# Autodesk Inventor assembly: quadcopter
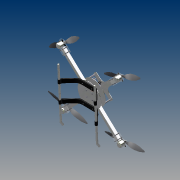
[picture p0: Inventor's stored thumbnail of the model, 180x180]
Saved by Autodesk Inventor 2011 SP1 (Build 150282100, 282)
## iProperties
Created: 2011-07-18
Part Number: quadcopter
Document SubType Name: Assembly
Designer: Nathan
Author: Nathan
## Documents named in this file (22)
- C:\Users\Nathan\Documents\Inventor\Quadcopter\quadcopter.iam
- C:\Users\Nathan\Documents\Inventor\Quadcopter\Arm.ipt
- C:\Users\Nathan\Documents\Inventor\Quadcopter\BaseTop.ipt
- C:\Users\Nathan\Documents\Inventor\Quadcopter\BaseBottom.ipt
- C:\Users\Nathan\Documents\Inventor\Quadcopter\MotorMount.iam
- C:\Users\Nathan\Documents\Inventor\Quadcopter\standoffiPart.ipt
- C:\Users\Nathan\Documents\Inventor\Quadcopter\standoffiPart-021.ipt
- C:\Users\Nathan\Documents\Inventor\Content Center Files\R2011\en-US\ANSI B18.6.3(26)\ANSI B18.6.3 - 8-32 UNC - 1.25(7).ipt
- C:\Users\Nathan\Documents\Inventor\Content Center Files\R2011\en-US\ANSI B18.6.3(26)\ANSI B18.6.3 - 8-32 UNC - 1.125(7).ipt
- C:\Users\Nathan\Documents\Inventor\Quadcopter\Imported Components\User Library-Arduino Mega\Assembly2.iam
- C:\Users\Nathan\Documents\Inventor\Quadcopter\LandingGear.iam
- C:\Users\Nathan\Documents\Inventor\Quadcopter\TopPlate.ipt
- C:\Users\Nathan\Documents\Inventor\Content Center Files\R2011\en-US\ANSI B18.6.3(26)\ANSI B18.6.3 - 8-32 UNC - 0.5(7).ipt
- C:\Users\Nathan\Documents\Inventor\Content Center Files\R2011\en-US\ANSI B18.6.3(26)\ANSI B18.6.3 - 4-40 UNC - 0.625(7).ipt
- C:\Users\Nathan\Documents\Inventor\Quadcopter\Motor.iam
- C:\Users\Nathan\Documents\Inventor\Quadcopter\propeller.iam
- C:\Users\Nathan\Documents\Inventor\Content Center Files\R2011\en-US\ANSI B18.6.3(26)\ANSI B18.6.3 - 6-32 UNC - 0.5625(7).ipt
- C:\Users\Nathan\Documents\Inventor\Quadcopter\PropProtector.ipt
- C:\Users\Nathan\Documents\Inventor\Content Center Files\R2011\en-US\ANSI B18.6.3(26)\ANSI B18.6.3 - 8-32 UNC - 1.375(7).ipt
- C:\Users\Nathan\Documents\Inventor\Content Center Files\R2011\en-US\ANSI B18.6.3(26)\ANSI B18.6.3 - 6-32 UNC - 0.5(7).ipt
- C:\Users\Nathan\Documents\Inventor\Quadcopter\Spacer_8-32.ipt
- C:\Users\Nathan\Documents\Inventor\Quadcopter\Spacer_4-40.ipt
## Components (58 placed, 20 different names)
1. Arm:1 — Mate:1, Mate:2, Mate:15, Flush:20, Mate:20, Flush:27, Mate:168, Mate:169
2. Arm:2 — Mate:5, Mate:6, Flush:21, Mate:21, Mate:38, Flush:25, Mate:160, Mate:161
3. Arm:3 — Mate:3, Mate:4, Flush:22, Mate:22, Flush:24, Mate:63, Mate:164, Mate:165
4. Arm:4 — Mate:7, Mate:8, Flush:23, Mate:23, Flush:26, Mate:78, Mate:97, Mate:157
5. BaseTop:1 — Mate:1, Mate:2, Mate:3, Mate:4, Mate:5, Mate:6, Mate:7, Mate:8, Mate:13, Mate:14, Mate:16, Mate:18, Mate:24, Mate:25, Mate:46, Mate:47, Mate:48, Mate:49, Mate:55, Mate:57, Mate:59, Mate:61, Angle:1, Mate:109, Mate:110, Mate:111, Mate:112, Flush:28, Flush:29, Mate:171, Mate:176, Mate:177, Mate:178, Mate:179
6. BaseBottom:1 — Mate:13, Mate:14, Mate:15, Mate:17, Mate:19, Mate:26, Mate:27, Mate:38, Mate:50, Mate:51, Mate:52, Mate:53, Mate:63, Mate:97, Mate:113, Mate:114, Mate:115, Mate:148, Mate:149, Mate:150, Mate:151, Mate:152, Mate:153, Mate:154, Mate:155, Mate:171
7. Cross Recessed Pan Head Machine Screw - Type II - Inch No. 8 - 32 - 1 1/4:1 — Mate:16, Mate:17, Mate:54, Mate:167
8. Cross Recessed Pan Head Machine Screw - Type II - Inch No. 8 - 32 - 1 1/8:2 — Mate:18, Mate:19, Mate:170
9. Cross Recessed Pan Head Machine Screw - Type II - Inch No. 8 - 32 - 1 1/4:7 — Mate:24, Mate:26, Mate:56, Mate:166
10. Cross Recessed Pan Head Machine Screw - Type II - Inch No. 8 - 32 - 1 1/8:3 — Mate:25, Mate:27, Mate:163
11. MotorMount:1 [sub-assembly] — Flush:20, Mate:20, Flush:27, Mate:136, Mate:137
12. MotorMount:2 [sub-assembly] — Flush:21, Mate:21, Flush:25, Mate:140, Mate:141
13. MotorMount:3 [sub-assembly] — Flush:22, Mate:22, Flush:24, Mate:142, Mate:143
14. MotorMount:4 [sub-assembly] — Flush:23, Mate:23, Flush:26, Mate:138, Mate:139
15. Cross Recessed Pan Head Machine Screw - Type II - Inch No. 8 - 32 - 1 3/8:1 — Mate:46, Mate:51, Mate:58, Mate:162
16. Cross Recessed Pan Head Machine Screw - Type II - Inch No. 8 - 32 - 1 1/8:4 — Mate:48, Mate:52, Mate:77
17. Cross Recessed Pan Head Machine Screw - Type II - Inch No. 8 - 32 - 1 1/4:2 — Mate:49, Mate:53, Mate:60, Mate:158
18. Cross Recessed Pan Head Machine Screw - Type II - Inch No. 8 - 32 - 1 1/8:1 — Mate:47, Mate:50, Mate:159
19. standoffiPart-021:5 — Mate:58, Mate:59, Mate:117, Mate:118
20. standoffiPart-021:6 — Mate:54, Mate:55
21. standoffiPart-021:7 — Mate:56, Mate:57
22. standoffiPart-021:8 — Mate:60, Mate:61, Mate:116
23. Spacer_8-32:1 — Mate:77, Mate:78
24. Assembly2:1 [sub-assembly] — Mate:103, Angle:1, Mate:105, Mate:106, Mate:107, Mate:108, Mate:180
25. Cross Recessed Pan Head Machine Screw - Type II - Inch No. 4 - 40 - 5/8:2 — Mate:107, Mate:109, Mate:175
26. Cross Recessed Pan Head Machine Screw - Type II - Inch No. 4 - 40 - 5/8:4 — Mate:106, Mate:112, Mate:174
27. Cross Recessed Pan Head Machine Screw - Type II - Inch No. 4 - 40 - 5/8:1 — Mate:103, Mate:108, Mate:111, Mate:172
28. Cross Recessed Pan Head Machine Screw - Type II - Inch No. 4 - 40 - 5/8:3 — Mate:105, Mate:110, Mate:173
29. LandingGear:1 [sub-assembly] — Mate:113, Mate:114, Mate:115
30. TopPlate:1 — Mate:116, Mate:117, Mate:118, Mate:119, Mate:120, Mate:121, Mate:122, Mate:123, Mate:124, Mate:125, Mate:126
31. Cross Recessed Pan Head Machine Screw - Type II - Inch No. 8 - 32 - 1/2:1 — Mate:119, Mate:126
32. Cross Recessed Pan Head Machine Screw - Type II - Inch No. 8 - 32 - 1/2:2 — Mate:120, Mate:123
33. Cross Recessed Pan Head Machine Screw - Type II - Inch No. 8 - 32 - 1/2:3 — Mate:122, Mate:124
34. Cross Recessed Pan Head Machine Screw - Type II - Inch No. 8 - 32 - 1/2:4 — Mate:121, Mate:125
35. Motor:1 [sub-assembly] — Mate:136, Mate:137, Mate:146
36. Motor:2 [sub-assembly] — Mate:140, Mate:141, Mate:145
37. Motor:3 [sub-assembly] — Mate:142, Mate:143, Mate:144, Mate:156
38. Motor:4 [sub-assembly] — Mate:138, Mate:139, Mate:147
39. propeller:1 [sub-assembly] — Mate:144
40. propeller:2 [sub-assembly] — Mate:145
41. propeller:3 [sub-assembly] — Mate:146
42. propeller:4 [sub-assembly] — Mate:147
43. Cross Recessed Pan Head Machine Screw - Type II - Inch No. 6 - 32 - 1/2:1 — Mate:148, Mate:149
44. Cross Recessed Pan Head Machine Screw - Type II - Inch No. 6 - 32 - 9/16:4 — Mate:154, Mate:155
45. Cross Recessed Pan Head Machine Screw - Type II - Inch No. 6 - 32 - 9/16:3 — Mate:152, Mate:153
46. Cross Recessed Pan Head Machine Screw - Type II - Inch No. 6 - 32 - 9/16:1 — Mate:150, Mate:151
47. PropProtector:1 — Flush:28, Flush:29, Mate:156
48. Spacer_8-32:2 — Mate:169, Mate:170
49. Spacer_8-32:3 — Mate:163, Mate:164
50. Spacer_8-32:4 — Mate:165, Mate:166
51. Spacer_8-32:5 — Mate:161, Mate:162
52. Spacer_8-32:6 — Mate:157, Mate:158
53. Spacer_8-32:7 — Mate:159, Mate:160
54. Spacer_8-32:8 — Mate:167, Mate:168
55. Spacer_4-40:1 — Mate:173, Mate:179
56. Spacer_4-40:2 — Mate:172, Mate:178, Mate:180
57. Spacer_4-40:3 — Mate:175, Mate:177
58. Spacer_4-40:4 — Mate:174, Mate:176
## Relationships (123: Mate 112, Flush 10, Angle 1)
- Mate:1: Arm:1 ↔ BaseTop:1
- Mate:2: Arm:1 ↔ BaseTop:1
- Mate:3: Arm:3 ↔ BaseTop:1
- Mate:4: Arm:3 ↔ BaseTop:1
- Mate:5: Arm:2 ↔ BaseTop:1
- Mate:6: Arm:2 ↔ BaseTop:1
- Mate:7: Arm:4 ↔ BaseTop:1
- Mate:8: Arm:4 ↔ BaseTop:1
- Mate:13: BaseTop:1 ↔ BaseBottom:1
- Mate:14: BaseTop:1 ↔ BaseBottom:1
- Mate:15: Arm:1 ↔ BaseBottom:1
- Mate:16: BaseTop:1 ↔ Cross Recessed Pan Head Machine Screw - Type II - Inch No. 8 - 32 - 1 1/4:1
- Mate:17: BaseBottom:1 ↔ Cross Recessed Pan Head Machine Screw - Type II - Inch No. 8 - 32 - 1 1/4:1
- Mate:18: BaseTop:1 ↔ Cross Recessed Pan Head Machine Screw - Type II - Inch No. 8 - 32 - 1 1/8:2
- Mate:19: BaseBottom:1 ↔ Cross Recessed Pan Head Machine Screw - Type II - Inch No. 8 - 32 - 1 1/8:2
- Flush:20: Arm:1 ↔ MotorMount:1
- Mate:20: Arm:1 ↔ MotorMount:1
- Flush:21: Arm:2 ↔ MotorMount:2
- Mate:21: Arm:2 ↔ MotorMount:2
- Flush:22: Arm:3 ↔ MotorMount:3
- Mate:22: Arm:3 ↔ MotorMount:3
- Flush:23: Arm:4 ↔ MotorMount:4
- Mate:23: Arm:4 ↔ MotorMount:4
- Mate:24: BaseTop:1 ↔ Cross Recessed Pan Head Machine Screw - Type II - Inch No. 8 - 32 - 1 1/4:7
- Mate:25: BaseTop:1 ↔ Cross Recessed Pan Head Machine Screw - Type II - Inch No. 8 - 32 - 1 1/8:3
- Mate:26: BaseBottom:1 ↔ Cross Recessed Pan Head Machine Screw - Type II - Inch No. 8 - 32 - 1 1/4:7
- Mate:27: BaseBottom:1 ↔ Cross Recessed Pan Head Machine Screw - Type II - Inch No. 8 - 32 - 1 1/8:3
- Mate:38: Arm:2 ↔ BaseBottom:1
- Flush:24: Arm:3 ↔ MotorMount:3
- Flush:25: Arm:2 ↔ MotorMount:2
- Flush:26: Arm:4 ↔ MotorMount:4
- Flush:27: Arm:1 ↔ MotorMount:1
- Mate:46: BaseTop:1 ↔ Cross Recessed Pan Head Machine Screw - Type II - Inch No. 8 - 32 - 1 3/8:1
- Mate:47: BaseTop:1 ↔ Cross Recessed Pan Head Machine Screw - Type II - Inch No. 8 - 32 - 1 1/8:1
- Mate:48: BaseTop:1 ↔ Cross Recessed Pan Head Machine Screw - Type II - Inch No. 8 - 32 - 1 1/8:4
- Mate:49: BaseTop:1 ↔ Cross Recessed Pan Head Machine Screw - Type II - Inch No. 8 - 32 - 1 1/4:2
- Mate:50: BaseBottom:1 ↔ Cross Recessed Pan Head Machine Screw - Type II - Inch No. 8 - 32 - 1 1/8:1
- Mate:51: BaseBottom:1 ↔ Cross Recessed Pan Head Machine Screw - Type II - Inch No. 8 - 32 - 1 3/8:1
- Mate:52: BaseBottom:1 ↔ Cross Recessed Pan Head Machine Screw - Type II - Inch No. 8 - 32 - 1 1/8:4
- Mate:53: BaseBottom:1 ↔ Cross Recessed Pan Head Machine Screw - Type II - Inch No. 8 - 32 - 1 1/4:2
- Mate:54: Cross Recessed Pan Head Machine Screw - Type II - Inch No. 8 - 32 - 1 1/4:1 ↔ standoffiPart-021:6
- Mate:55: BaseTop:1 ↔ standoffiPart-021:6
- Mate:56: Cross Recessed Pan Head Machine Screw - Type II - Inch No. 8 - 32 - 1 1/4:7 ↔ standoffiPart-021:7
- Mate:57: BaseTop:1 ↔ standoffiPart-021:7
- Mate:58: Cross Recessed Pan Head Machine Screw - Type II - Inch No. 8 - 32 - 1 3/8:1 ↔ standoffiPart-021:5
- Mate:59: BaseTop:1 ↔ standoffiPart-021:5
- Mate:60: Cross Recessed Pan Head Machine Screw - Type II - Inch No. 8 - 32 - 1 1/4:2 ↔ standoffiPart-021:8
- Mate:61: BaseTop:1 ↔ standoffiPart-021:8
- Mate:63: Arm:3 ↔ BaseBottom:1
- Mate:77: Cross Recessed Pan Head Machine Screw - Type II - Inch No. 8 - 32 - 1 1/8:4 ↔ Spacer_8-32:1
- Mate:78: Arm:4 ↔ Spacer_8-32:1
- Mate:97: Arm:4 ↔ BaseBottom:1
- Mate:103: Assembly2:1 ↔ Cross Recessed Pan Head Machine Screw - Type II - Inch No. 4 - 40 - 5/8:1
- Angle:1 (0 deg): BaseTop:1 ↔ Assembly2:1
- Mate:105: Assembly2:1 ↔ Cross Recessed Pan Head Machine Screw - Type II - Inch No. 4 - 40 - 5/8:3
- Mate:106: Assembly2:1 ↔ Cross Recessed Pan Head Machine Screw - Type II - Inch No. 4 - 40 - 5/8:4
- Mate:107: Assembly2:1 ↔ Cross Recessed Pan Head Machine Screw - Type II - Inch No. 4 - 40 - 5/8:2
- Mate:108: Assembly2:1 ↔ Cross Recessed Pan Head Machine Screw - Type II - Inch No. 4 - 40 - 5/8:1
- Mate:109: BaseTop:1 ↔ Cross Recessed Pan Head Machine Screw - Type II - Inch No. 4 - 40 - 5/8:2
- Mate:110: BaseTop:1 ↔ Cross Recessed Pan Head Machine Screw - Type II - Inch No. 4 - 40 - 5/8:3
- Mate:111: BaseTop:1 ↔ Cross Recessed Pan Head Machine Screw - Type II - Inch No. 4 - 40 - 5/8:1
- Mate:112: BaseTop:1 ↔ Cross Recessed Pan Head Machine Screw - Type II - Inch No. 4 - 40 - 5/8:4
- Mate:113: BaseBottom:1 ↔ LandingGear:1
- Mate:114: BaseBottom:1 ↔ LandingGear:1
- Mate:115 (3.175 mm): BaseBottom:1 ↔ LandingGear:1
- Mate:116: standoffiPart-021:8 ↔ TopPlate:1
- Mate:117: standoffiPart-021:5 ↔ TopPlate:1
- Mate:118: standoffiPart-021:5 ↔ TopPlate:1
- Mate:119: TopPlate:1 ↔ Cross Recessed Pan Head Machine Screw - Type II - Inch No. 8 - 32 - 1/2:1
- Mate:120: TopPlate:1 ↔ Cross Recessed Pan Head Machine Screw - Type II - Inch No. 8 - 32 - 1/2:2
- Mate:121: TopPlate:1 ↔ Cross Recessed Pan Head Machine Screw - Type II - Inch No. 8 - 32 - 1/2:4
- Mate:122: TopPlate:1 ↔ Cross Recessed Pan Head Machine Screw - Type II - Inch No. 8 - 32 - 1/2:3
- Mate:123: TopPlate:1 ↔ Cross Recessed Pan Head Machine Screw - Type II - Inch No. 8 - 32 - 1/2:2
- Mate:124: TopPlate:1 ↔ Cross Recessed Pan Head Machine Screw - Type II - Inch No. 8 - 32 - 1/2:3
- Mate:125: TopPlate:1 ↔ Cross Recessed Pan Head Machine Screw - Type II - Inch No. 8 - 32 - 1/2:4
- Mate:126: TopPlate:1 ↔ Cross Recessed Pan Head Machine Screw - Type II - Inch No. 8 - 32 - 1/2:1
- Mate:136: MotorMount:1 ↔ Motor:1
- Mate:137: MotorMount:1 ↔ Motor:1
- Mate:138: MotorMount:4 ↔ Motor:4
- Mate:139: MotorMount:4 ↔ Motor:4
- Mate:140: MotorMount:2 ↔ Motor:2
- Mate:141: MotorMount:2 ↔ Motor:2
- Mate:142: MotorMount:3 ↔ Motor:3
- Mate:143: MotorMount:3 ↔ Motor:3
- Mate:144: Motor:3 ↔ propeller:1
- Mate:145: Motor:2 ↔ propeller:2
- Mate:146: Motor:1 ↔ propeller:3
- Mate:147: Motor:4 ↔ propeller:4
- Mate:148: BaseBottom:1 ↔ Cross Recessed Pan Head Machine Screw - Type II - Inch No. 6 - 32 - 1/2:1
- Mate:149: BaseBottom:1 ↔ Cross Recessed Pan Head Machine Screw - Type II - Inch No. 6 - 32 - 1/2:1
- Mate:150: BaseBottom:1 ↔ Cross Recessed Pan Head Machine Screw - Type II - Inch No. 6 - 32 - 9/16:1
- Mate:151: BaseBottom:1 ↔ Cross Recessed Pan Head Machine Screw - Type II - Inch No. 6 - 32 - 9/16:1
- Mate:152: BaseBottom:1 ↔ Cross Recessed Pan Head Machine Screw - Type II - Inch No. 6 - 32 - 9/16:3
- Mate:153: BaseBottom:1 ↔ Cross Recessed Pan Head Machine Screw - Type II - Inch No. 6 - 32 - 9/16:3
- Mate:154: BaseBottom:1 ↔ Cross Recessed Pan Head Machine Screw - Type II - Inch No. 6 - 32 - 9/16:4
- Mate:155: BaseBottom:1 ↔ Cross Recessed Pan Head Machine Screw - Type II - Inch No. 6 - 32 - 9/16:4
- Flush:28: BaseTop:1 ↔ PropProtector:1
- Flush:29: BaseTop:1 ↔ PropProtector:1
- Mate:156: Motor:3 ↔ PropProtector:1
- Mate:157: Arm:4 ↔ Spacer_8-32:6
- Mate:158: Cross Recessed Pan Head Machine Screw - Type II - Inch No. 8 - 32 - 1 1/4:2 ↔ Spacer_8-32:6
- Mate:159: Cross Recessed Pan Head Machine Screw - Type II - Inch No. 8 - 32 - 1 1/8:1 ↔ Spacer_8-32:7
- Mate:160: Arm:2 ↔ Spacer_8-32:7
- Mate:161: Arm:2 ↔ Spacer_8-32:5
- Mate:162: Cross Recessed Pan Head Machine Screw - Type II - Inch No. 8 - 32 - 1 3/8:1 ↔ Spacer_8-32:5
- Mate:163: Cross Recessed Pan Head Machine Screw - Type II - Inch No. 8 - 32 - 1 1/8:3 ↔ Spacer_8-32:3
- Mate:164: Arm:3 ↔ Spacer_8-32:3
- Mate:165: Arm:3 ↔ Spacer_8-32:4
- Mate:166: Cross Recessed Pan Head Machine Screw - Type II - Inch No. 8 - 32 - 1 1/4:7 ↔ Spacer_8-32:4
- Mate:167: Cross Recessed Pan Head Machine Screw - Type II - Inch No. 8 - 32 - 1 1/4:1 ↔ Spacer_8-32:8
- Mate:168: Arm:1 ↔ Spacer_8-32:8
- Mate:169: Arm:1 ↔ Spacer_8-32:2
- Mate:170: Cross Recessed Pan Head Machine Screw - Type II - Inch No. 8 - 32 - 1 1/8:2 ↔ Spacer_8-32:2
- Mate:171 (22.225 mm): BaseTop:1 ↔ BaseBottom:1
- Mate:172: Cross Recessed Pan Head Machine Screw - Type II - Inch No. 4 - 40 - 5/8:1 ↔ Spacer_4-40:2
- Mate:173: Cross Recessed Pan Head Machine Screw - Type II - Inch No. 4 - 40 - 5/8:3 ↔ Spacer_4-40:1
- Mate:174: Cross Recessed Pan Head Machine Screw - Type II - Inch No. 4 - 40 - 5/8:4 ↔ Spacer_4-40:4
- Mate:175: Cross Recessed Pan Head Machine Screw - Type II - Inch No. 4 - 40 - 5/8:2 ↔ Spacer_4-40:3
- Mate:176: BaseTop:1 ↔ Spacer_4-40:4
- Mate:177: BaseTop:1 ↔ Spacer_4-40:3
- Mate:178: BaseTop:1 ↔ Spacer_4-40:2
- Mate:179: BaseTop:1 ↔ Spacer_4-40:1
- Mate:180: Assembly2:1 ↔ Spacer_4-40:2
